# Autodesk Inventor assembly: MM3
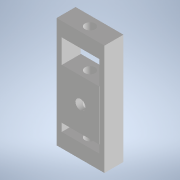
[picture p0: Inventor's stored thumbnail of the model, 180x180]
Saved by Autodesk Inventor 2021 (Build 250183000, 183)
## iProperties
Created: 2021-02-23
Part Number: MM3
Document SubType Name: Assembly
Designer: dsdan
Author: dsdan
## Documents named in this file (3)
- E:\OneDrive - Imperial College London\DragonVision_DanielKo\Instrumentation\Ephys_rig_2021\MM3.iam
- E:\OneDrive - Imperial College London\DragonVision_DanielKo\Instrumentation\Ephys_rig_2021\MM3_track.ipt
- E:\OneDrive - Imperial College London\DragonVision_DanielKo\Instrumentation\Ephys_rig_2021\MM3_cage.ipt
## Components (2 placed, 2 different names)
1. MM3_track:1 — Flush:1, Mate:1
2. MM3_cage:1 — Flush:1, Mate:1
## Relationships (2: Flush 1, Mate 1)
- Flush:1: MM3_track:1 ↔ MM3_cage:1
- Mate:1: MM3_track:1 ↔ MM3_cage:1
